# Autodesk Inventor assembly: Assembly
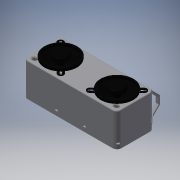
[picture p0: Inventor's stored thumbnail of the model, 180x180]
Saved by Autodesk Inventor 2016 (Build 200138000, 138)
## iProperties
Created: 2019-09-19
Part Number: Assembly
Document SubType Name: Assembly
Designer: jimmy
Author: jimmy
## Documents named in this file (10)
- D:\DS Cloud\Projects\Portable speaker\CADs\Assembly.iam
- D:\DS Cloud\Projects\Portable speaker\CADs\Housing.ipt
- D:\DS Cloud\Projects\Portable speaker\CADs\Speaker_Massive_MX3.ipt
- D:\DS Cloud\Projects\Portable speaker\CADs\PCB\PCB.iam
- D:\DS Cloud\Projects\Portable speaker\CADs\Battery_LI polymer_30C.ipt
- D:\DS Cloud\Projects\Portable speaker\CADs\Fan bracket.ipt
- D:\DS Cloud\Projects\Portable speaker\CADs\Fan.ipt
- D:\DS Cloud\Projects\Portable speaker\CADs\USB plug.ipt
- D:\DS Cloud\Projects\Portable speaker\CADs\Switch_DC_Pilot.ipt
- D:\DS Cloud\Projects\Portable speaker\CADs\Housing cover.ipt
## Components (11 placed, 9 different names)
1. Housing:1 — Mate:1, Mate:2, Mate:3, Mate:4, Tangent:1, Tangent:2, Mate:7, Mate:8, Mate:9, Mate:10, Mate:11, Mate:13, Mate:14, Insert:1, Insert:2, Insert:3, Mate:18, Mate:19, Mate:20
2. Speaker_Massive_MX3:1 — Mate:3, Mate:4, Tangent:2
3. Speaker_Massive_MX3:2 — Mate:1, Mate:2, Tangent:1
4. Battery_LI polymer_30C:1 — Mate:7, Mate:8
5. PCB:1 [sub-assembly] — Mate:9, Mate:10, Mate:11, Mate:12
6. Fan bracket:1 — Mate:12, Mate:13, Mate:14, Mate:15, Mate:16, Mate:17
7. Fan:1 — Mate:15, Mate:16, Mate:17
8. USB plug:1 — Insert:1
9. Switch_DC_Pilot:1 — Insert:2
10. Switch_DC_Pilot:2 — Insert:3
11. Housing cover:1 — Mate:18, Mate:19, Mate:20
## Relationships (23: Mate 18, Insert 3, Tangent 2)
- Mate:1: Housing:1 ↔ Speaker_Massive_MX3:2
- Mate:2: Housing:1 ↔ Speaker_Massive_MX3:2
- Mate:3: Housing:1 ↔ Speaker_Massive_MX3:1
- Mate:4: Housing:1 ↔ Speaker_Massive_MX3:1
- Tangent:1: Housing:1 ↔ Speaker_Massive_MX3:2
- Tangent:2: Housing:1 ↔ Speaker_Massive_MX3:1
- Mate:7: Housing:1 ↔ Battery_LI polymer_30C:1
- Mate:8: Housing:1 ↔ Battery_LI polymer_30C:1
- Mate:9: Housing:1 ↔ PCB:1
- Mate:10: Housing:1 ↔ PCB:1
- Mate:11: Housing:1 ↔ PCB:1
- Mate:12: PCB:1 ↔ Fan bracket:1
- Mate:13: Housing:1 ↔ Fan bracket:1
- Mate:14: Housing:1 ↔ Fan bracket:1
- Mate:15: Fan bracket:1 ↔ Fan:1
- Mate:16: Fan bracket:1 ↔ Fan:1
- Mate:17: Fan bracket:1 ↔ Fan:1
- Insert:1: Housing:1 ↔ USB plug:1
- Insert:2: Housing:1 ↔ Switch_DC_Pilot:1
- Insert:3: Housing:1 ↔ Switch_DC_Pilot:2
- Mate:18: Housing:1 ↔ Housing cover:1
- Mate:19: Housing:1 ↔ Housing cover:1
- Mate:20: Housing:1 ↔ Housing cover:1
